# Autodesk Inventor assembly: Assembly1
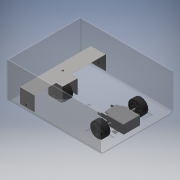
[picture p0: Inventor's stored thumbnail of the model, 180x180]
Saved by Autodesk Inventor 2019 (Build 230136000, 136)
## iProperties
Created: 2019-08-08
Part Number: Assembly1
Document SubType Name: Assembly
Designer: daozhou.cen
Author: daozhou.cen
## Documents named in this file (12)
- P:\Composite\All Students\Robotics Club\Bowen\Maze Navigation Robot\Design\Assembly1.iam
- P:\Composite\All Students\Robotics Club\Bowen\Maze Navigation Robot\Design\Part1.ipt
- P:\Composite\All Students\Robotics Club\Bowen\Maze Navigation Robot\Design\Part2.ipt
- P:\Composite\All Students\Robotics Club\Bowen\Maze Navigation Robot\Design\Part3.ipt
- P:\Composite\All Students\Robotics Club\Bowen\Maze Navigation Robot\Design\Part4.ipt
- P:\Composite\All Students\Robotics Club\Bowen\Maze Navigation Robot\Design\Part5.ipt
- P:\Composite\All Students\Robotics Club\Bowen\Maze Navigation Robot\Design\Part6.ipt
- P:\Composite\All Students\Robotics Club\Bowen\Maze Navigation Robot\Design\Part7.ipt
- P:\Composite\All Students\Robotics Club\Bowen\Maze Navigation Robot\Design\Part8.ipt
- P:\Composite\All Students\Robotics Club\Bowen\Maze Navigation Robot\Design\Part9.ipt
- P:\Composite\All Students\Robotics Club\Bowen\Maze Navigation Robot\Design\Part10.ipt
- P:\Composite\All Students\Robotics Club\Bowen\Maze Navigation Robot\Design\Part11.ipt
## Components (33 placed, 11 different names)
1. Part1:1 — Rigid:2
2. Part1:2 — Rigid:1
3. Part2:1 — Rigid:1, Rigid:2, Rigid:5, Rotational:18, Rotational:21, Rotational:24, Rotational:25
4. Part3:1 — Rotational:3, Rotational:7, Rotational:8
5. Part3:2 — Rotational:1, Rotational:10, Rotational:12
6. Part3:3 — Rotational:2, Rotational:9, Rotational:11
7. Part4:1 — Rotational:1, Rotational:2, Rotational:24, Rotational:25, Rigid:6, Rigid:7
8. Part5:1 — Rotational:3, Cylindrical:1, Mate:1
9. Part6:1 — Cylindrical:1, Rotational:4, Rotational:5, Rotational:6, Rigid:3, Rotational:13, Rotational:14, Mate:1
10. Part7:4 — Rotational:4
11. Part7:5 — Rotational:6
12. Part7:6 — Rotational:5
13. Part7:7 — Rigid:3
14. Part7:8 — Rotational:8
15. Part7:9 — Rotational:7
16. Part7:10 — Rotational:12
17. Part7:11 — Rotational:11
18. Part7:12 — Rotational:10
19. Part7:13 — Rotational:9
20. Part8:1 — Rotational:15, Rotational:17
21. Part7:14 — Rotational:13, Rotational:15
22. Part7:15 — Rotational:14
23. Part9:1 — Rigid:4, Rigid:5, Rotational:20, Rotational:23
24. Part7:16 — Rotational:16
25. Part7:17 — Rigid:4, Rotational:16, Rotational:17
26. Part10:1 — Rotational:19
27. Part10:2 — Rotational:22
28. Part7:18 — Rotational:18, Rotational:19
29. Part7:19 — Rotational:20
30. Part7:20 — Rotational:21, Rotational:22
31. Part7:21 — Rotational:23
32. Part11:1 — Rigid:6
33. Part11:2 — Rigid:7
## Relationships (34: RevoluteJoint 25, WeldJoint 7, CylindricalJoint 1, Mate 1)
- Rigid:1 [WeldJoint]: Part1:2 ↔ Part2:1
- Rigid:2 [WeldJoint]: Part1:1 ↔ Part2:1
- Rotational:1 [RevoluteJoint] (-1 mm): Part3:2 ↔ Part4:1
- Rotational:2 [RevoluteJoint] (-1 mm): Part3:3 ↔ Part4:1
- Rotational:3 [RevoluteJoint] (5 mm): Part3:1 ↔ Part5:1
- Cylindrical:1: Part5:1 ↔ Part6:1
- Rotational:4 [RevoluteJoint]: Part6:1 ↔ Part7:4
- Rotational:5 [RevoluteJoint]: Part6:1 ↔ Part7:6
- Rotational:6 [RevoluteJoint]: Part6:1 ↔ Part7:5
- Rigid:3 [WeldJoint]: Part6:1 ↔ Part7:7
- Rotational:7 [RevoluteJoint]: Part3:1 ↔ Part7:9
- Rotational:8 [RevoluteJoint]: Part3:1 ↔ Part7:8
- Rotational:9 [RevoluteJoint]: Part3:3 ↔ Part7:13
- Rotational:10 [RevoluteJoint]: Part3:2 ↔ Part7:12
- Rotational:11 [RevoluteJoint]: Part3:3 ↔ Part7:11
- Rotational:12 [RevoluteJoint]: Part3:2 ↔ Part7:10
- Rotational:13 [RevoluteJoint]: Part6:1 ↔ Part7:14
- Rotational:14 [RevoluteJoint]: Part6:1 ↔ Part7:15
- Rotational:15 [RevoluteJoint]: Part8:1 ↔ Part7:14
- Rigid:4 [WeldJoint]: Part9:1 ↔ Part7:17
- Rotational:16 [RevoluteJoint]: Part7:16 ↔ Part7:17
- Rotational:17 [RevoluteJoint]: Part8:1 ↔ Part7:17
- Rigid:5 [WeldJoint]: Part2:1 ↔ Part9:1
- Mate:1 (5 mm): Part5:1 ↔ Part6:1
- Rotational:18 [RevoluteJoint]: Part2:1 ↔ Part7:18
- Rotational:19 [RevoluteJoint]: Part10:1 ↔ Part7:18
- Rotational:20 [RevoluteJoint]: Part9:1 ↔ Part7:19
- Rotational:21 [RevoluteJoint]: Part2:1 ↔ Part7:20
- Rotational:22 [RevoluteJoint]: Part10:2 ↔ Part7:20
- Rotational:23 [RevoluteJoint]: Part9:1 ↔ Part7:21
- Rotational:24 [RevoluteJoint]: Part2:1 ↔ Part4:1
- Rotational:25 [RevoluteJoint]: Part2:1 ↔ Part4:1
- Rigid:6 [WeldJoint] (-1 mm): Part4:1 ↔ Part11:1
- Rigid:7 [WeldJoint] (-1 mm): Part4:1 ↔ Part11:2
